# Autodesk Inventor assembly: arm_MIR
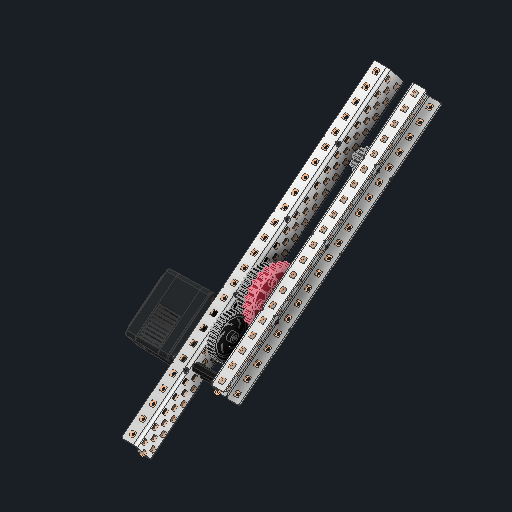
[picture p0: Inventor's stored thumbnail of the model, 512x512]
Saved by Autodesk Inventor 2024 (Build 280153000, 153)
## iProperties
Created: 2023-10-22
Part Number: arm_MIR
Document SubType Name: Assembly
Designer: Averey Ku
Author: Averey Ku
## Documents named in this file (9)
- D:\vex_robotics\hardware\cad\spades_v0.1\intake\mirrored_parts\arm_MIR.iam
- D:\vex_robotics\hardware\cad\spades_v0.1\intake\mirrored_parts\Alu C 1x2x1x25_MIR.ipt
- D:\vex_robotics\hardware\cad\spades_v0.1\intake\mirrored_parts\V5 Motor (5.5W)_MIR.ipt
- D:\vex_robotics\hardware\cad\spades_v0.1\intake\mirrored_parts\Alu C 1x2x1x20_MIR.ipt
- D:\vex_robotics\hardware\cad\spades_v0.1\intake\mirrored_parts\LS 36T Gear_MIR.ipt
- D:\vex_robotics\hardware\cad\spades_v0.1\intake\mirrored_parts\6P 24T Sprocket, No Insert_MIR.iam
- D:\vex_robotics\hardware\cad\spades_v0.1\intake\mirrored_parts\6P 8T Sprocket, No Insert_MIR.iam
- D:\vex_robotics\hardware\cad\VEX-CAD-Inventor-1.41\Structure\Standoff\Standoff .875.ipt
- D:\vex_robotics\hardware\cad\VEX-CAD-Inventor-1.41\Structure\Standoff.ipt
## Components (9 placed, 7 different names)
1. Alu C 1x2x1x25_MIR:1 — Insert:2, Insert:9, Insert:14, Insert:15
2. V5 Motor (5.5W)_MIR:1
3. Alu C 1x2x1x20_MIR:1 — Insert:13, Insert:16, Mate:1
4. LS 36T Gear_MIR:1 — Insert:2
5. LS 36T Gear_MIR:2 — Insert:9, Insert:10
6. 6P 24T Sprocket, No Insert_MIR:1 [sub-assembly] — Insert:10
7. 6P 8T Sprocket, No Insert_MIR:1 [sub-assembly] — Insert:13
8. Standoff .875:1 — Insert:16, Insert:14
9. Standoff .875:2 — Mate:1, Insert:15
## Relationships (8: Insert 7, Mate 1)
- Insert:2: Alu C 1x2x1x25_MIR:1 ↔ LS 36T Gear_MIR:1
- Insert:9: Alu C 1x2x1x25_MIR:1 ↔ LS 36T Gear_MIR:2
- Insert:10: LS 36T Gear_MIR:2 ↔ 6P 24T Sprocket, No Insert_MIR:1
- Insert:13: Alu C 1x2x1x20_MIR:1 ↔ 6P 8T Sprocket, No Insert_MIR:1
- Insert:16: Alu C 1x2x1x20_MIR:1 ↔ Standoff .875:1
- Insert:14: Alu C 1x2x1x25_MIR:1 ↔ Standoff .875:1
- Mate:1: Alu C 1x2x1x20_MIR:1 ↔ Standoff .875:2
- Insert:15: Alu C 1x2x1x25_MIR:1 ↔ Standoff .875:2
